# Autodesk Inventor assembly: Fertige_Baugruppe
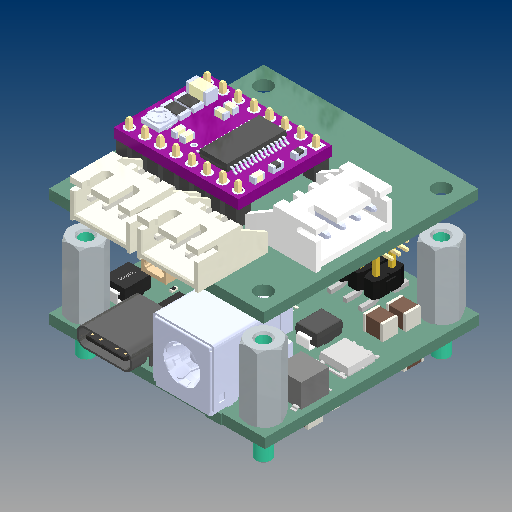
[picture p0: Inventor's stored thumbnail of the model, 512x512]
Saved by Autodesk Inventor 2025 (Build 290162010, 162A)
## iProperties
Created: 2025-02-26
Part Number: Fertige_Baugruppe
Document SubType Name: Assembly
Designer: jan
Author: jan
## Documents named in this file (3)
- C:\Users\jan\Documents\github\fiberprinter-electronics\2nd-mainboard-pcb\export_versions\Fertige_Baugruppe.iam
- C:\Users\jan\Documents\github\fiberprinter-electronics\2nd-mainboard-pcb\export_versions\V1\V1.iam
- C:\Users\jan\Documents\github\fiberprinter-electronics\2nd-mainboard-pcb\export_versions\V2\V1.iam
## Components (2 placed, 1 different names)
1. V1:1 [sub-assembly] — Passend:1, Passend:2
2. V1:2 [sub-assembly] — Passend:1, Passend:2
## Relationships (2: Mate 2)
- Passend:1 [Mate]: V1:1 ↔ V1:2
- Passend:2 [Mate]: V1:1 ↔ V1:2
